# Autodesk Inventor assembly: Final_Assembly
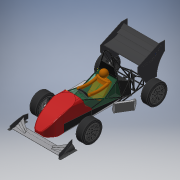
[picture p0: Inventor's stored thumbnail of the model, 180x180]
Saved by Autodesk Inventor 2018.1 (Build 221171000, 171)
## iProperties
Created: 2017-11-02
Part Number: Final_Assembly
Material: 一般
Document SubType Name: Assembly
Designer: kuwano
Author: kuwano
## Documents named in this file (4)
- D:\kuwano\Documents\Inventor\KITformula\AeroCAD2018\CAD\Inventor\Final_Assembly.iam
- D:\kuwano\Documents\Inventor\KITformula\AeroCAD2018\CAD\Inventor\Assembly(KS-14.ver)\KS-14_SLow\KS-14_SLow_replace.iam
- D:\kuwano\Documents\Inventor\KITformula\AeroCAD2018\CAD\Inventor\Aero Parts\F-wing\type6\F-wing.iam
- D:\kuwano\Documents\Inventor\KITformula\AeroCAD2018\CAD\Inventor\Aero Parts\R-wing\type6\R-wing.iam
## Components (3 placed, 3 different names)
1. KS-14_SLow_replace:1 [sub-assembly] — メイト:1, メイト:2, メイト:3, メイト:4
2. F-wing:1 [sub-assembly] — フラッシュ:1, メイト:4, フラッシュ:2
3. R-wing:1 [sub-assembly] — フラッシュ:3
## Relationships (7: Mate 4, Flush 3)
- メイト:1 [Mate]: KS-14_SLow_replace:1
- メイト:2 [Mate]: KS-14_SLow_replace:1
- メイト:3 [Mate]: KS-14_SLow_replace:1
- フラッシュ:1 [Flush]: F-wing:1
- メイト:4 [Mate] (400 mm): KS-14_SLow_replace:1 ↔ F-wing:1
- フラッシュ:2 [Flush] (-250 mm): F-wing:1
- フラッシュ:3 [Flush]: R-wing:1
